# Autodesk Inventor assembly: Payload and Box
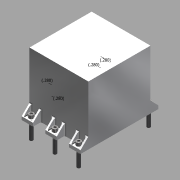
[picture p0: Inventor's stored thumbnail of the model, 180x180]
Saved by Autodesk Inventor 2017 (Build 210142000, 142)
## iProperties
Created: 2017-02-16
Part Number: Payload and Box
Document SubType Name: Assembly
Designer: qupec
Author: qupec
## Documents named in this file (4)
- C:\Users\qupec\Desktop\UMD Near Space\STAR\CAD\Mechanical\Payload and Box.iam
- C:\Users\qupec\Desktop\UMD Near Space\STAR\CAD\Mechanical\Full payload assembly.iam
- C:\Users\qupec\Desktop\UMD Near Space\STAR\CAD\Mechanical\Payload Box.ipt
- C:\Users\qupec\Documents\Inventor\Content Center Files\R2017\en-US\U UNC 2603(1)\Unbrako - 1_4 x 1 1_2 - 28 - 1.5 - Unbrako.ipt
## Components (8 placed, 3 different names)
1. Full payload assembly:1 [sub-assembly] — Mate:1, Mate:2, Flush:1
2. Payload Box:1 — Mate:1, Mate:2, Flush:1, Mate:3, Mate:4, Mate:5, Mate:6, Mate:7, Mate:8, Mate:9, Mate:10, Mate:11, Mate:12, Mate:13, Mate:14
3. Unbrako UNC Hex Socket Cap - Inch 1/4 x 1 1/2 - Unbrako:1 — Mate:8, Mate:10
4. Unbrako UNC Hex Socket Cap - Inch 1/4 x 1 1/2 - Unbrako:2 — Mate:6, Mate:11
5. Unbrako UNC Hex Socket Cap - Inch 1/4 x 1 1/2 - Unbrako:3 — Mate:3, Mate:14
6. Unbrako UNC Hex Socket Cap - Inch 1/4 x 1 1/2 - Unbrako:4 — Mate:7, Mate:9
7. Unbrako UNC Hex Socket Cap - Inch 1/4 x 1 1/2 - Unbrako:5 — Mate:5, Mate:12
8. Unbrako UNC Hex Socket Cap - Inch 1/4 x 1 1/2 - Unbrako:6 — Mate:4, Mate:13
## Relationships (15: Mate 14, Flush 1)
- Mate:1: Full payload assembly:1 ↔ Payload Box:1
- Mate:2: Full payload assembly:1 ↔ Payload Box:1
- Flush:1: Full payload assembly:1 ↔ Payload Box:1
- Mate:3: Payload Box:1 ↔ Unbrako UNC Hex Socket Cap - Inch 1/4 x 1 1/2 - Unbrako:3
- Mate:4: Payload Box:1 ↔ Unbrako UNC Hex Socket Cap - Inch 1/4 x 1 1/2 - Unbrako:6
- Mate:5: Payload Box:1 ↔ Unbrako UNC Hex Socket Cap - Inch 1/4 x 1 1/2 - Unbrako:5
- Mate:6: Payload Box:1 ↔ Unbrako UNC Hex Socket Cap - Inch 1/4 x 1 1/2 - Unbrako:2
- Mate:7: Payload Box:1 ↔ Unbrako UNC Hex Socket Cap - Inch 1/4 x 1 1/2 - Unbrako:4
- Mate:8: Payload Box:1 ↔ Unbrako UNC Hex Socket Cap - Inch 1/4 x 1 1/2 - Unbrako:1
- Mate:9: Payload Box:1 ↔ Unbrako UNC Hex Socket Cap - Inch 1/4 x 1 1/2 - Unbrako:4
- Mate:10: Payload Box:1 ↔ Unbrako UNC Hex Socket Cap - Inch 1/4 x 1 1/2 - Unbrako:1
- Mate:11: Payload Box:1 ↔ Unbrako UNC Hex Socket Cap - Inch 1/4 x 1 1/2 - Unbrako:2
- Mate:12: Payload Box:1 ↔ Unbrako UNC Hex Socket Cap - Inch 1/4 x 1 1/2 - Unbrako:5
- Mate:13: Payload Box:1 ↔ Unbrako UNC Hex Socket Cap - Inch 1/4 x 1 1/2 - Unbrako:6
- Mate:14: Payload Box:1 ↔ Unbrako UNC Hex Socket Cap - Inch 1/4 x 1 1/2 - Unbrako:3
